# Autodesk Inventor assembly: XY Joint Left (Tulip)
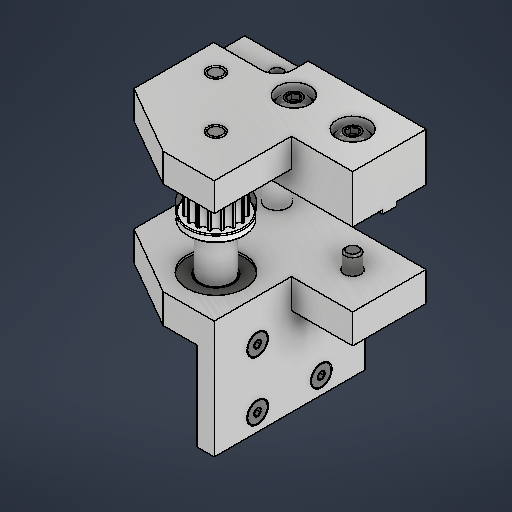
[picture p0: Inventor's stored thumbnail of the model, 512x512]
Saved by Autodesk Inventor 2026 (Build 300175050, 175E)
## iProperties
Created: 2025-05-24
Part Number: XY Joint Left (Tulip)
Document SubType Name: Assembly
Designer: Joshua Eah
Author: Joshua Eah
## Documents named in this file (14)
- C:\Users\Joshua Eah\Documents\GitHub\Voron-0\CAD\Tulip - Machined Parts\XY Joint Left\XY Joint Left (Tulip).iam
- C:\Users\Joshua Eah\Documents\GitHub\Voron-0\CAD\Tulip - Machined Parts\XY Joint Left\XY Joint Left Upper (Tulip).ipt
- C:\Users\Joshua Eah\Documents\GitHub\Voron-0\CAD\Tulip - Machined Parts\XY Joint Left\XY Joint Left Lower (Tulip).ipt
- C:\Users\Joshua Eah\Documents\GitHub\Voron-0\CAD\Master Assembly\Hardware\f623-rs.ipt
- C:\Users\Joshua Eah\Documents\GitHub\Voron-0\CAD\Master Assembly\Hardware\M3_Washer.ipt
- C:\Users\Joshua Eah\Documents\GitHub\Voron-0\CAD\Tulip - Machined Parts\Spacers\Live Idler Spacer.ipt
- C:\Users\Joshua Eah\Documents\GitHub\Voron-0\CAD\Master Assembly\Hardware\3x30 Pin.ipt
- C:\Users\Joshua Eah\Documents\GitHub\Voron-0\CAD\Master Assembly\Hardware\F623 Stack.iam
- C:\Users\Joshua Eah\Documents\GitHub\Voron-0\CAD\Machined Parts\Spacers\Spacer.ipt
- C:\Users\Joshua Eah\Documents\GitHub\Voron-0\CAD\Master Assembly\Hardware\M3x6 BHCS.ipt
- C:\Users\Joshua Eah\Documents\GitHub\Voron-0\CAD\Master Assembly\Hardware\M3x12 BHCS.ipt
- C:\Users\Joshua Eah\Documents\GitHub\Voron-0\CAD\Master Assembly\Hardware\M2x6 FHCS.ipt
- C:\Users\Joshua Eah\Documents\GitHub\Voron-0\CAD\Tulip - Machined Parts\Spacers\Joint Spacer.ipt
- C:\Users\Joshua Eah\Documents\GitHub\Voron-0\CAD\Master Assembly\Hardware\16T_Pulley.ipt
## Components (21 placed, 13 different names)
1. XY Joint Left Upper (Tulip):1 — Insert:2, Insert:13, Insert:14, Insert:19, Insert:20
2. XY Joint Left Lower (Tulip):1 — Insert:1, Mate:1, Mate:2, Mate:7, Insert:12, Insert:15, Insert:16, Insert:17, Insert:18
3. f623-rs:1 — Insert:1, Insert:11
4. f623-rs:2 — Insert:2, Insert:4, Mate:5
5. M3_Washer:2 — Insert:4
6. Live Idler Spacer:1 — Insert:6, Insert:11
7. 16T_Pulley:1 — Insert:6, Mate:8
8. 3x30 Pin:1 — Mate:1, Mate:2, Flush:1, Mate:6
9. F623 Stack:1 [sub-assembly] — Insert:8, Insert:9, Mate:6
10. M3_Washer:3 — Insert:8, Mate:7
11. M3_Washer:4 — Insert:9, Insert:10
12. 3x30 Pin:2 — Mate:5, Flush:1, Mate:8
13. Spacer:1 — Insert:10, Insert:20
14. M3x6 BHCS:1 — Insert:12
15. M3x12 BHCS:1 — Insert:13
16. M3x12 BHCS:2 — Insert:14
17. M2x6 FHCS:1 — Insert:15
18. M2x6 FHCS:2 — Insert:16
19. M2x6 FHCS:3 — Insert:17
20. M2x6 FHCS:4 — Insert:18
21. Joint Spacer:1 — Insert:19
## Relationships (24: Insert 17, Mate 6, Flush 1)
- Insert:1: XY Joint Left Lower (Tulip):1 ↔ f623-rs:1
- Insert:2: XY Joint Left Upper (Tulip):1 ↔ f623-rs:2
- Insert:4: f623-rs:2 ↔ M3_Washer:2
- Insert:6: Live Idler Spacer:1 ↔ 16T_Pulley:1
- Mate:1: XY Joint Left Lower (Tulip):1 ↔ 3x30 Pin:1
- Mate:2: XY Joint Left Lower (Tulip):1 ↔ 3x30 Pin:1
- Mate:5: f623-rs:2 ↔ 3x30 Pin:2
- Flush:1: 3x30 Pin:1 ↔ 3x30 Pin:2
- Insert:8: F623 Stack:1 ↔ M3_Washer:3
- Insert:9: F623 Stack:1 ↔ M3_Washer:4
- Mate:6: 3x30 Pin:1 ↔ F623 Stack:1
- Mate:7: XY Joint Left Lower (Tulip):1 ↔ M3_Washer:3
- Insert:10: M3_Washer:4 ↔ Spacer:1
- Insert:11: f623-rs:1 ↔ Live Idler Spacer:1
- Insert:12: XY Joint Left Lower (Tulip):1 ↔ M3x6 BHCS:1
- Insert:13: XY Joint Left Upper (Tulip):1 ↔ M3x12 BHCS:1
- Insert:14: XY Joint Left Upper (Tulip):1 ↔ M3x12 BHCS:2
- Insert:15: XY Joint Left Lower (Tulip):1 ↔ M2x6 FHCS:1
- Insert:16: XY Joint Left Lower (Tulip):1 ↔ M2x6 FHCS:2
- Insert:17: XY Joint Left Lower (Tulip):1 ↔ M2x6 FHCS:3
- Insert:18: XY Joint Left Lower (Tulip):1 ↔ M2x6 FHCS:4
- Insert:19: XY Joint Left Upper (Tulip):1 ↔ Joint Spacer:1
- Insert:20: XY Joint Left Upper (Tulip):1 ↔ Spacer:1
- Mate:8: 16T_Pulley:1 ↔ 3x30 Pin:2
